# Autodesk Inventor assembly: sensor-temperatura
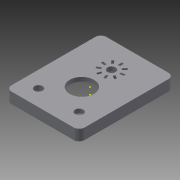
[picture p0: Inventor's stored thumbnail of the model, 180x180]
Saved by Autodesk Inventor 2015 SP1 (Build 190203100, 203)
## iProperties
Created: 2015-07-05
Part Number: sensor-temperatura
Document SubType Name: Assembly
Designer: Javier
Author: Javier
## Documents named in this file (4)
- D:\Dropbox\3dprint\riego\sensores\sensor-temperatura.iam
- D:\Dropbox\3dprint\riego\sensores\base.ipt
- D:\Dropbox\3dprint\riego\sensores\temperatura.ipt
- D:\Dropbox\3dprint\riego\sensores\luz.ipt
## Components (3 placed, 3 different names)
1. base:1 — Nivelación:1
2. temperatura:1 — Nivelación:1
3. luz:1
## Relationships (1: Flush 1)
- Nivelación:1 [Flush]: base:1 ↔ temperatura:1
